# Autodesk Inventor assembly: MAIN
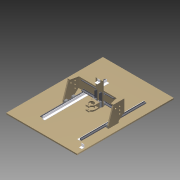
[picture p0: Inventor's stored thumbnail of the model, 180x180]
Saved by Autodesk Inventor 2012 (Build 160160000, 160)
## iProperties
Created: 2013-05-09
Part Number: MAIN
Document SubType Name: Assembly
Designer: Fabian
Author: Fabian
## Documents named in this file (14)
- E:\Users\Fabian\Documents\Autodesk\Projects\CNC Router\MAIN.iam
- E:\Users\Fabian\Documents\Autodesk\Projects\Laser cutter\rail long.ipt
- E:\Users\Fabian\Documents\Autodesk\Projects\Laser cutter\new baseboard.ipt
- E:\Users\Fabian\Documents\Autodesk\Projects\Laser cutter\Linear bearing.ipt
- E:\Users\Fabian\Documents\Autodesk\Projects\CNC Router\angle support.ipt
- E:\Users\Fabian\Documents\Autodesk\Projects\CNC Router\Uprights.ipt
- E:\Users\Fabian\Documents\Autodesk\Projects\CNC Router\back crossboard.ipt
- E:\Users\Fabian\Documents\Autodesk\Projects\Laser cutter\rail short.ipt
- E:\Users\Fabian\Documents\Autodesk\Projects\CNC Router\Z plate.ipt
- E:\Users\Fabian\Documents\Autodesk\Projects\CNC Router\z rail.ipt
- E:\Users\Fabian\Documents\Autodesk\Projects\CNC Router\Router mount.ipt
- E:\Users\Fabian\Documents\Autodesk\Projects\CNC Router\z moving plate.ipt
- E:\Users\Fabian\Documents\Autodesk\Projects\Laser cutter\stepper motor bracket.ipt
- E:\Users\Fabian\Documents\Autodesk\Projects\CNC Router\ridgidizer.ipt
## Components (32 placed, 13 different names)
1. rail long:1 — Mate:3, Flush:4, Flush:5, Mate:7, Mate:8
2. rail long:2 — Mate:4, Flush:6, Flush:7, Mate:5, Mate:6
3. new baseboard:1 — Mate:1, Mate:2, Flush:1, Flush:3, Mate:42, Flush:49
4. Linear bearing:1 — Mate:8, Flush:8, Mate:9, Flush:12, Mate:11
5. Linear bearing:2 — Mate:7, Flush:8, Mate:9, Flush:11
6. Linear bearing:3 — Mate:6, Flush:9, Mate:10, Flush:13, Flush:14
7. Linear bearing:4 — Mate:5, Flush:9, Mate:10, Mate:12
8. angle support:1 — Mate:1, Flush:2, Flush:3, Mate:4, Flush:6, Flush:7
9. angle support:2 — Mate:2, Flush:1, Flush:2, Mate:3, Flush:4, Flush:5
10. Uprights:1 — Flush:11, Flush:12, Mate:11, Flush:15, Flush:16, Flush:17, Flush:18, Mate:18
11. Uprights:2 — Mate:12, Flush:13, Flush:14, Flush:15, Flush:16, Mate:13, Flush:19, Flush:20
12. back crossboard:1 — Mate:13, Flush:17, Flush:18, Flush:19, Flush:20, Mate:16, Mate:17, Mate:43, Flush:47, Flush:48, Flush:51, Mate:45, Flush:52, Flush:53
13. rail short:1 — Mate:17, Flush:24, Mate:20, Mate:22, Flush:48
14. rail short:2 — Mate:16, Mate:18, Flush:24, Mate:19, Mate:21
15. Linear bearing:5 — Flush:25, Mate:20, Flush:29, Flush:30
16. Linear bearing:6 — Flush:25, Flush:26, Flush:27, Mate:21, Flush:29, Mate:23, Mate:24, Flush:31, Flush:51
17. Linear bearing:7 — Flush:26, Mate:19, Flush:28, Mate:23
18. Linear bearing:8 — Flush:27, Mate:22, Flush:28
19. Z plate:1 — Flush:30, Mate:24, Flush:31, Mate:25, Mate:26, Flush:32, Flush:33, Flush:34, Flush:35, Mate:44, Flush:50, Flush:54
20. z rail:1 — Mate:25, Flush:32, Flush:33, Mate:27, Mate:30
21. z rail:2 — Mate:26, Flush:34, Flush:35, Mate:28, Mate:29
22. Linear bearing:9 — Mate:27, Flush:37, Flush:38, Flush:39
23. Linear bearing:10 — Mate:28, Flush:37, Flush:39, Mate:31, Flush:41, Flush:42
24. Linear bearing:11 — Mate:30, Flush:36, Flush:38, Flush:40
25. Linear bearing:12 — Mate:29, Flush:36, Flush:40, Mate:31, Mate:32
26. Router mount:1 — Mate:33, Flush:43, Flush:44
27. Router mount:2 — Mate:34, Flush:45, Flush:46
28. z moving plate:1 — Mate:32, Flush:41, Flush:42, Mate:33, Flush:43, Flush:44, Mate:34, Flush:45, Flush:46
29. stepper motor bracket:1 — Mate:44, Flush:50, Flush:54
30. stepper motor bracket:2 — Mate:43, Flush:47
31. stepper motor bracket:3 — Mate:42, Flush:49
32. ridgidizer:1 — Mate:45, Flush:52, Flush:53
## Relationships (86: Flush 50, Mate 36)
- Mate:1: new baseboard:1 ↔ angle support:1
- Mate:2: new baseboard:1 ↔ angle support:2
- Flush:1 (152.4 mm): new baseboard:1 ↔ angle support:2
- Flush:2: angle support:1 ↔ angle support:2
- Flush:3 (304.8 mm): new baseboard:1 ↔ angle support:1
- Mate:3: rail long:1 ↔ angle support:2
- Flush:4: rail long:1 ↔ angle support:2
- Flush:5: rail long:1 ↔ angle support:2
- Mate:4: rail long:2 ↔ angle support:1
- Flush:6: rail long:2 ↔ angle support:1
- Flush:7: rail long:2 ↔ angle support:1
- Mate:5: rail long:2 ↔ Linear bearing:4
- Mate:6: rail long:2 ↔ Linear bearing:3
- Mate:7: rail long:1 ↔ Linear bearing:2
- Mate:8: rail long:1 ↔ Linear bearing:1
- Flush:8: Linear bearing:1 ↔ Linear bearing:2
- Flush:9: Linear bearing:3 ↔ Linear bearing:4
- Mate:9 (76.2 mm): Linear bearing:1 ↔ Linear bearing:2
- Mate:10 (76.2 mm): Linear bearing:3 ↔ Linear bearing:4
- Flush:11: Linear bearing:2 ↔ Uprights:1
- Flush:12: Linear bearing:1 ↔ Uprights:1
- Mate:11: Linear bearing:1 ↔ Uprights:1
- Mate:12: Linear bearing:4 ↔ Uprights:2
- Flush:13: Linear bearing:3 ↔ Uprights:2
- Flush:14: Linear bearing:3 ↔ Uprights:2
- Flush:15: Uprights:1 ↔ Uprights:2
- Flush:16: Uprights:1 ↔ Uprights:2
- Mate:13: Uprights:2 ↔ back crossboard:1
- Flush:17: Uprights:1 ↔ back crossboard:1
- Flush:18: Uprights:1 ↔ back crossboard:1
- Flush:19: Uprights:2 ↔ back crossboard:1
- Flush:20: Uprights:2 ↔ back crossboard:1
- Mate:16: back crossboard:1 ↔ rail short:2
- Mate:17: back crossboard:1 ↔ rail short:1
- Mate:18 (101.6 mm): Uprights:1 ↔ rail short:2
- Flush:24: rail short:1 ↔ rail short:2
- Flush:25: Linear bearing:5 ↔ Linear bearing:6
- Flush:26: Linear bearing:6 ↔ Linear bearing:7
- Flush:27: Linear bearing:6 ↔ Linear bearing:8
- Mate:19: rail short:2 ↔ Linear bearing:7
- Mate:20: rail short:1 ↔ Linear bearing:5
- Mate:21: rail short:2 ↔ Linear bearing:6
- Mate:22: rail short:1 ↔ Linear bearing:8
- Flush:28: Linear bearing:7 ↔ Linear bearing:8
- Flush:29: Linear bearing:5 ↔ Linear bearing:6
- Mate:23 (25.4 mm): Linear bearing:6 ↔ Linear bearing:7
- Flush:30: Linear bearing:5 ↔ Z plate:1
- Mate:24: Linear bearing:6 ↔ Z plate:1
- Flush:31 (-165.1 mm): Linear bearing:6 ↔ Z plate:1
- Mate:25: Z plate:1 ↔ z rail:1
- Mate:26: Z plate:1 ↔ z rail:2
- Flush:32: Z plate:1 ↔ z rail:1
- Flush:33 (-152.4 mm): Z plate:1 ↔ z rail:1
- Flush:34 (152.4 mm): Z plate:1 ↔ z rail:2
- Flush:35: Z plate:1 ↔ z rail:2
- Mate:27: z rail:1 ↔ Linear bearing:9
- Mate:28: z rail:2 ↔ Linear bearing:10
- Mate:29: z rail:2 ↔ Linear bearing:12
- Mate:30: z rail:1 ↔ Linear bearing:11
- Flush:36: Linear bearing:11 ↔ Linear bearing:12
- Flush:37: Linear bearing:9 ↔ Linear bearing:10
- Flush:38: Linear bearing:9 ↔ Linear bearing:11
- Flush:39: Linear bearing:9 ↔ Linear bearing:10
- Flush:40: Linear bearing:11 ↔ Linear bearing:12
- Mate:31: Linear bearing:10 ↔ Linear bearing:12
- Mate:32: Linear bearing:12 ↔ z moving plate:1
- Flush:41: Linear bearing:10 ↔ z moving plate:1
- Flush:42: Linear bearing:10 ↔ z moving plate:1
- Mate:33: Router mount:1 ↔ z moving plate:1
- Flush:43: Router mount:1 ↔ z moving plate:1
- Flush:44: Router mount:1 ↔ z moving plate:1
- Mate:34: Router mount:2 ↔ z moving plate:1
- Flush:45: Router mount:2 ↔ z moving plate:1
- Flush:46: Router mount:2 ↔ z moving plate:1
- Mate:42: new baseboard:1 ↔ stepper motor bracket:3
- Mate:43: back crossboard:1 ↔ stepper motor bracket:2
- Flush:47 (76.2 mm): back crossboard:1 ↔ stepper motor bracket:2
- Flush:48: back crossboard:1 ↔ rail short:1
- Flush:49 (25.4 mm): new baseboard:1 ↔ stepper motor bracket:3
- Mate:44: Z plate:1 ↔ stepper motor bracket:1
- Flush:50: Z plate:1 ↔ stepper motor bracket:1
- Flush:51 (2.54 mm): back crossboard:1 ↔ Linear bearing:6
- Mate:45: back crossboard:1 ↔ ridgidizer:1
- Flush:52: back crossboard:1 ↔ ridgidizer:1
- Flush:53: back crossboard:1 ↔ ridgidizer:1
- Flush:54 (31.75 mm): Z plate:1 ↔ stepper motor bracket:1
